# Autodesk Inventor assembly: Main Body - Full Assembly
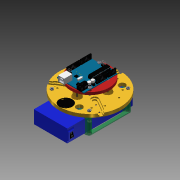
[picture p0: Inventor's stored thumbnail of the model, 180x180]
Saved by Autodesk Inventor 2014 (Build 180170000, 170)
## iProperties
Created: 2014-02-14
Part Number: Main Body - Full Assembly
Document SubType Name: Assembly
Designer: Spooner
Author: Spooner
## Documents named in this file (14)
- C:\Users\Spooner\Documents\Inventor\FerretBall Robot\3Pod\Inventor 2014 Files\Main Body - Full Assembly.iam
- C:\Users\Spooner\Documents\Inventor\FerretBall Robot\3Pod\Inventor 2014 Files\Arduino Mount.ipt
- C:\Users\Spooner\Documents\Inventor\FerretBall Robot\3Pod\Inventor 2014 Files\Body.ipt
- C:\Users\Spooner\Documents\Inventor\FerretBall Robot\3Pod\Inventor 2014 Files\Gyro Mount.ipt
- C:\Users\Spooner\Documents\Inventor\FerretBall Robot\3Pod\Inventor 2014 Files\Offset.ipt
- C:\Users\Spooner\Documents\Inventor\Content Center Files\R2014\en-US\JIS B 1111(1)\JIS B 1111 - M3x30(1).ipt
- C:\Users\Spooner\Documents\Inventor\Content Center Files\R2014\en-US\JIS B 1181 U\JIS B 1181 - B M3.ipt
- C:\Users\Spooner\Documents\Inventor\FerretBall Robot\3Pod\Inventor 2014 Files\Arduino.ipt
- C:\Users\Spooner\Documents\Inventor\Content Center Files\R2014\en-US\JIS B 1111(1)\JIS B 1111 - M3x12(1).ipt
- C:\Users\Spooner\Documents\Inventor\FerretBall Robot\3Pod\Inventor 2014 Files\12 Volt Battery Pack.ipt
- C:\Users\Spooner\Documents\Inventor\FerretBall Robot\3Pod\Inventor 2014 Files\Battery Holder Top.ipt
- C:\Users\Spooner\Documents\Inventor\FerretBall Robot\3Pod\Inventor 2014 Files\Battery Holder Bottom.ipt
- C:\Users\Spooner\Documents\Inventor\Content Center Files\R2014\en-US\JIS B 1111(1)\JIS B 1111 - M3x20(1).ipt
- C:\Users\Spooner\Documents\Inventor\Content Center Files\R2014\en-US\JIS B 1111(1)\JIS B 1111 - M3x40(1).ipt
## Components (32 placed, 13 different names)
1. Arduino Mount:1 — Insert:6, Insert:7, Insert:8, Insert:9, Insert:10, Insert:14, Mate:1, Insert:19, Insert:20, Insert:21, Insert:22
2. Body:1 — Insert:1, Insert:2, Insert:3, Insert:11, Insert:12, Insert:13, Insert:29, Insert:30, Insert:31, Insert:32
3. Gyro Mount:1 — Insert:4, Insert:5, Insert:6, Insert:7
4. Offset:1 — Insert:3, Insert:5
5. Offset:2 — Insert:2, Insert:4
6. Offset:3 — Insert:1
7. JIS B 1111 M3x40:1 — Insert:8, Mate:3
8. JIS B 1111 M3x40:2 — Insert:9
9. JIS B 1111 M3x30:3 — Insert:10
10. JIS B 1181 (unchamfered) - Metric B M3:1 — Insert:11
11. JIS B 1181 (unchamfered) - Metric B M3:2 — Insert:12, Insert:23
12. JIS B 1181 (unchamfered) - Metric B M3:3 — Insert:13
13. Arduino:1 — Insert:14, Mate:1, Insert:15, Insert:16, Insert:17, Insert:18
14. JIS B 1111 M3x12:3 — Insert:15
15. JIS B 1111 M3x12:1 — Insert:18
16. JIS B 1111 M3x12:2 — Insert:16
17. JIS B 1111 M3x12:4 — Insert:17
18. JIS B 1181 (unchamfered) - Metric B M3:4 — Insert:22
19. JIS B 1181 (unchamfered) - Metric B M3:5 — Insert:21
20. JIS B 1181 (unchamfered) - Metric B M3:6 — Insert:20
21. JIS B 1181 (unchamfered) - Metric B M3:7 — Insert:19
22. 12 Volt Battery Pack:1 — Mate:5, Mate:6, Mate:8, Mate:9
23. Battery Holder Top:1 — Insert:23, Mate:3, Mate:5, Mate:6, Insert:24, Mate:7, Mate:8
24. Battery Holder Bottom:1 — Insert:24, Mate:7, Insert:25, Mate:9, Insert:26, Insert:27, Insert:28
25. JIS B 1111 M3x20:5 — Insert:25
26. JIS B 1111 M3x20:2 — Insert:28
27. JIS B 1111 M3x20:3 — Insert:26
28. JIS B 1111 M3x20:4 — Insert:27
29. JIS B 1181 (unchamfered) - Metric B M3:8 — Insert:29
30. JIS B 1181 (unchamfered) - Metric B M3:9 — Insert:32
31. JIS B 1181 (unchamfered) - Metric B M3:10 — Insert:31
32. JIS B 1181 (unchamfered) - Metric B M3:11 — Insert:30
## Relationships (39: Insert 32, Mate 7)
- Insert:1: Body:1 ↔ Offset:3
- Insert:2: Body:1 ↔ Offset:2
- Insert:3: Body:1 ↔ Offset:1
- Insert:4: Gyro Mount:1 ↔ Offset:2
- Insert:5: Gyro Mount:1 ↔ Offset:1
- Insert:6: Arduino Mount:1 ↔ Gyro Mount:1
- Insert:7: Arduino Mount:1 ↔ Gyro Mount:1
- Insert:8: Arduino Mount:1 ↔ JIS B 1111 M3x40:1
- Insert:9: Arduino Mount:1 ↔ JIS B 1111 M3x40:2
- Insert:10: Arduino Mount:1 ↔ JIS B 1111 M3x30:3
- Insert:11: Body:1 ↔ JIS B 1181 (unchamfered) - Metric B M3:1
- Insert:12: Body:1 ↔ JIS B 1181 (unchamfered) - Metric B M3:2
- Insert:13: Body:1 ↔ JIS B 1181 (unchamfered) - Metric B M3:3
- Insert:14: Arduino Mount:1 ↔ Arduino:1
- Mate:1: Arduino Mount:1 ↔ Arduino:1
- Insert:15: Arduino:1 ↔ JIS B 1111 M3x12:3
- Insert:16: Arduino:1 ↔ JIS B 1111 M3x12:2
- Insert:17: Arduino:1 ↔ JIS B 1111 M3x12:4
- Insert:18: Arduino:1 ↔ JIS B 1111 M3x12:1
- Insert:19: Arduino Mount:1 ↔ JIS B 1181 (unchamfered) - Metric B M3:7
- Insert:20: Arduino Mount:1 ↔ JIS B 1181 (unchamfered) - Metric B M3:6
- Insert:21: Arduino Mount:1 ↔ JIS B 1181 (unchamfered) - Metric B M3:5
- Insert:22: Arduino Mount:1 ↔ JIS B 1181 (unchamfered) - Metric B M3:4
- Insert:23: JIS B 1181 (unchamfered) - Metric B M3:2 ↔ Battery Holder Top:1
- Mate:3: JIS B 1111 M3x40:1 ↔ Battery Holder Top:1
- Mate:5: 12 Volt Battery Pack:1 ↔ Battery Holder Top:1
- Mate:6: 12 Volt Battery Pack:1 ↔ Battery Holder Top:1
- Insert:24: Battery Holder Top:1 ↔ Battery Holder Bottom:1
- Mate:7: Battery Holder Top:1 ↔ Battery Holder Bottom:1
- Insert:25: Battery Holder Bottom:1 ↔ JIS B 1111 M3x20:5
- Mate:8: 12 Volt Battery Pack:1 ↔ Battery Holder Top:1
- Mate:9: 12 Volt Battery Pack:1 ↔ Battery Holder Bottom:1
- Insert:26: Battery Holder Bottom:1 ↔ JIS B 1111 M3x20:3
- Insert:27: Battery Holder Bottom:1 ↔ JIS B 1111 M3x20:4
- Insert:28: Battery Holder Bottom:1 ↔ JIS B 1111 M3x20:2
- Insert:29: Body:1 ↔ JIS B 1181 (unchamfered) - Metric B M3:8
- Insert:30: Body:1 ↔ JIS B 1181 (unchamfered) - Metric B M3:11
- Insert:31: Body:1 ↔ JIS B 1181 (unchamfered) - Metric B M3:10
- Insert:32: Body:1 ↔ JIS B 1181 (unchamfered) - Metric B M3:9
